# Autodesk Inventor assembly: Omniwheel
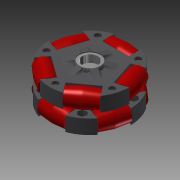
[picture p0: Inventor's stored thumbnail of the model, 180x180]
Saved by Autodesk Inventor 2014 SP2 (Build 180246200, 246)
## iProperties
Created: 2019-06-15
Part Number: Omniwheel
Document SubType Name: Assembly
Designer: Yuchofif
Author: Yuchofif
## Documents named in this file (4)
- D:\Inventor\Ofif\Suciman\Omniwheel\Omni Wheel Encoder\Omniwheel.iam
- D:\Inventor\Ofif\Suciman\Omniwheel\Omni Wheel Encoder\Cassing.ipt
- D:\Inventor\Ofif\Suciman\Omniwheel\Omni Wheel Encoder\Shaft.ipt
- D:\Inventor\Ofif\Suciman\Omniwheel\Omni Wheel Encoder\Rubber.ipt
## Components (13 placed, 3 different names)
1. Cassing:1 — Insert:1, Insert:2, Insert:3, Insert:4, Insert:5, Insert:6
2. Shaft:1 — Insert:1, Insert:7
3. Rubber:1 — Insert:3
4. Rubber:2 — Insert:2
5. Rubber:3 — Insert:6
6. Rubber:4 — Insert:5
7. Rubber:5 — Insert:4
8. Cassing:2 — Insert:7, Insert:8, Insert:9, Insert:10, Insert:11, Insert:12
9. Rubber:6 — Insert:8
10. Rubber:7 — Insert:10
11. Rubber:8 — Insert:9
12. Rubber:9 — Insert:11
13. Rubber:10 — Insert:12
## Relationships (12: Insert 12)
- Insert:1 (-35 mm): Cassing:1 ↔ Shaft:1
- Insert:2: Cassing:1 ↔ Rubber:2
- Insert:3: Cassing:1 ↔ Rubber:1
- Insert:4: Cassing:1 ↔ Rubber:5
- Insert:5: Cassing:1 ↔ Rubber:4
- Insert:6: Cassing:1 ↔ Rubber:3
- Insert:7 (22 mm): Shaft:1 ↔ Cassing:2
- Insert:8: Cassing:2 ↔ Rubber:6
- Insert:9: Cassing:2 ↔ Rubber:8
- Insert:10: Cassing:2 ↔ Rubber:7
- Insert:11: Cassing:2 ↔ Rubber:9
- Insert:12: Cassing:2 ↔ Rubber:10
